# Autodesk Inventor assembly: Сборка модуля
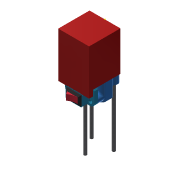
[picture p0: Inventor's stored thumbnail of the model, 180x180]
Saved by Autodesk Inventor 2022 (Build 260153000, 153)
## iProperties
Created: 2023-02-18
Part Number: Сборка модуля
Document SubType Name: Assembly
Designer: Ivan
Mass: 28.0565 g
Surface Area: 336.743 cm^2
Volume: 28.0565 cm^3
Density: 1 g/cm^3
Author: Ivan
## Documents named in this file (4)
- C:\Теплица\Сборка модуля.iam
- C:\Модуль\Сборка МК.iam
- C:\Модуль\Сборка АКБ.iam
- C:\Модуль\крышка для воздуха.ipt
## Components (3 placed, 3 different names)
1. Сборка МК:1 [sub-assembly] — Заподлицо:2, Заподлицо:3, Совмещение:1
2. Сборка АКБ:1 [sub-assembly] — Угол:1, Заподлицо:2, Заподлицо:3, Совмещение:1, Совмещение:4
3. крышка для воздуха:1 — Совмещение:4
## Relationships (5: Flush 2, Mate 2, Angle 1)
- Угол:1 [Angle] (180 deg): Сборка АКБ:1
- Заподлицо:2 [Flush]: Сборка МК:1 ↔ Сборка АКБ:1
- Заподлицо:3 [Flush]: Сборка МК:1 ↔ Сборка АКБ:1
- Совмещение:1 [Mate]: Сборка МК:1 ↔ Сборка АКБ:1
- Совмещение:4 [Mate]: Сборка АКБ:1 ↔ крышка для воздуха:1
